# Autodesk Inventor assembly: REV Ultraplanetary Motor 2 Cartridges
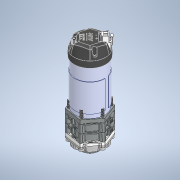
[picture p0: Inventor's stored thumbnail of the model, 180x180]
Saved by Autodesk Inventor 2022 (Build 260153000, 153)
## iProperties
Created: 2019-08-05
Part Number: REV Ultraplanetary Motor 2 Cartridges
Description: STEP AP214
Document SubType Name: Assembly
Designer: TakeHomePC
Sending System: SolidWorks 2018
Preprocessor: SwSTEP 2.0
Title: REV-41-1600.STEP
Revision Number: ANY
## Documents named in this file (9)
- C:\Users\matt\Documents\Inventor\FTC\2022-23 FTC\Motors\REV Ultraplanetary Motor 2 Cartridges.iam
- C:\Users\matt\Documents\Inventor\FTC\2022-23 FTC\Motors\REV-41-1301 No Gearbox_Without Gearbox.iam
- C:\Users\matt\Documents\Inventor\FTC\2022-23 FTC\Motors\REV-41-1607.ipt
- C:\Users\matt\Documents\Inventor\FTC\2022-23 FTC\Motors\M3x8 Button Head_91239A113.ipt
- C:\Users\matt\Documents\Inventor\FTC\2022-23 FTC\Motors\REV-41-1608.ipt
- C:\Users\matt\Documents\Inventor\FTC\2022-23 FTC\Motors\REV-41-1603.iam
- C:\Users\matt\Documents\Inventor\FTC\2022-23 FTC\Motors\REV-41-1602.iam
- C:\Users\matt\Documents\Inventor\FTC\2022-23 FTC\Motors\REV-41-1604.iam
- C:\Users\matt\Documents\Inventor\FTC\2022-23 FTC\Motors\M3X40_91290A136.ipt
## Components (14 placed, 14 different names)
1. REV-41-1301 No Gearbox_Without Gearbox_1 [sub-assembly] — Mate:20, Mate:22
2. REV-41-1607_2 — Mate:16, Mate:17, Mate:18, Mate:20, Mate:22
3. M3x8 Button Head_91239A113_3
4. REV-41-1608_4
5. REV-41-1603_5 [sub-assembly] — Mate:15, Mate:18, Mate:19, Mate:21
6. REV-41-1602_6 [sub-assembly] — Mate:1, Mate:14, Mate:19, Mate:23
7. M3x8 Button Head_91239A113_8
8. REV-41-1604_9 [sub-assembly] — Mate:1, Mate:2, Mate:3, Mate:4, Mate:5, Mate:6, Mate:7, Mate:8, Mate:9, Mate:10, Mate:11, Mate:12, Mate:13
9. M3X40_91290A136_10 — Mate:2, Mate:3, Mate:14, Mate:15, Mate:17
10. M3X40_91290A136_11 — Mate:5, Mate:12
11. M3X40_91290A136_12 — Mate:7, Mate:10
12. M3X40_91290A136_13 — Mate:4, Mate:13, Mate:16
13. M3X40_91290A136_14 — Mate:6, Mate:11, Mate:21, Mate:23
14. M3X40_91290A136_15 — Mate:8, Mate:9
## Relationships (23: Mate 23)
- Mate:1: REV-41-1602_6 ↔ REV-41-1604_9
- Mate:2: REV-41-1604_9 ↔ M3X40_91290A136_10
- Mate:3: REV-41-1604_9 ↔ M3X40_91290A136_10
- Mate:4: REV-41-1604_9 ↔ M3X40_91290A136_13
- Mate:5: REV-41-1604_9 ↔ M3X40_91290A136_11
- Mate:6: REV-41-1604_9 ↔ M3X40_91290A136_14
- Mate:7: REV-41-1604_9 ↔ M3X40_91290A136_12
- Mate:8: REV-41-1604_9 ↔ M3X40_91290A136_15
- Mate:9: REV-41-1604_9 ↔ M3X40_91290A136_15
- Mate:10: REV-41-1604_9 ↔ M3X40_91290A136_12
- Mate:11: REV-41-1604_9 ↔ M3X40_91290A136_14
- Mate:12: REV-41-1604_9 ↔ M3X40_91290A136_11
- Mate:13: REV-41-1604_9 ↔ M3X40_91290A136_13
- Mate:14: REV-41-1602_6 ↔ M3X40_91290A136_10
- Mate:15: REV-41-1603_5 ↔ M3X40_91290A136_10
- Mate:16: REV-41-1607_2 ↔ M3X40_91290A136_13
- Mate:17: REV-41-1607_2 ↔ M3X40_91290A136_10
- Mate:18: REV-41-1607_2 ↔ REV-41-1603_5
- Mate:19: REV-41-1603_5 ↔ REV-41-1602_6
- Mate:20: REV-41-1301 No Gearbox_Without Gearbox_1 ↔ REV-41-1607_2
- Mate:21: REV-41-1603_5 ↔ M3X40_91290A136_14
- Mate:22: REV-41-1301 No Gearbox_Without Gearbox_1 ↔ REV-41-1607_2
- Mate:23: REV-41-1602_6 ↔ M3X40_91290A136_14
